# Autodesk Inventor assembly: servo_leg_top_frame_with_nuts
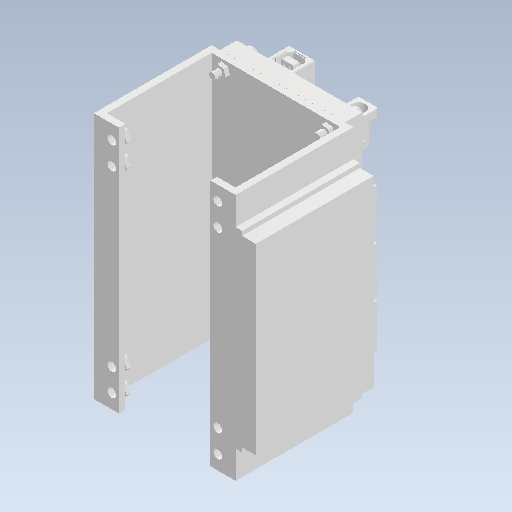
[picture p0: Inventor's stored thumbnail of the model, 512x512]
Saved by Autodesk Inventor 2021.4 (Build 254397000, 397)
## iProperties
Created: 2022-07-27
Part Number: servo_leg_top_frame_with_nuts
Document SubType Name: Assembly
Designer: isamu
Author: isamu
## Documents named in this file (4)
- D:\personal_projects\robot\inventor\2021_matlab_compat _v2\servo_frames\servo_leg_top_frame_with_nuts.iam
- D:\personal_projects\robot\inventor\2021_matlab_compat _v2\servo_frames\arduino_with_case.iam
- D:\personal_projects\robot\exports\breadboard.ipt
- D:\personal_projects\robot\inventor\2021_matlab_compat _v2\servo_frames\servo_leg_top_frame_with_nuts_without_arduino.iam
## Components (3 placed, 3 different names)
1. arduino_with_case:1 [sub-assembly] — Mate:1, Mate:2, Mate:3
2. breadboard:1 — Mate:4, Mate:5, Mate:6
3. servo_leg_top_frame_with_nuts_without_arduino:1 [sub-assembly] — Mate:1, Mate:2, Mate:3, Mate:4, Mate:5, Mate:6
## Relationships (6: Mate 6)
- Mate:1: arduino_with_case:1 ↔ servo_leg_top_frame_with_nuts_without_arduino:1
- Mate:2: arduino_with_case:1 ↔ servo_leg_top_frame_with_nuts_without_arduino:1
- Mate:3: arduino_with_case:1 ↔ servo_leg_top_frame_with_nuts_without_arduino:1
- Mate:4: breadboard:1 ↔ servo_leg_top_frame_with_nuts_without_arduino:1
- Mate:5: breadboard:1 ↔ servo_leg_top_frame_with_nuts_without_arduino:1
- Mate:6: breadboard:1 ↔ servo_leg_top_frame_with_nuts_without_arduino:1
